# Autodesk Inventor assembly: mount_camera_static
Saved by Autodesk Inventor 2021 (Build 250183000, 183)
## iProperties
Created: 2021-03-20
Part Number: mount_camera_static
Document SubType Name: Assembly
Designer: Tomasz Lisowski
Author: Tomasz Lisowski
## Documents named in this file (5)
- T:\repos\tcodev\tco-cad\mount_camera_static\mount_camera_static.iam
- T:\repos\tcodev\tco-cad\mount_camera_static\mount_camera_static_base.ipt
- T:\repos\tcodev\tco-cad\common\coral_camera.ipt
- T:\repos\tcodev\tco-cad\common\hardware\m2_standoff_6mm.ipt
- T:\repos\tcodev\tco-cad\common\hardware\m2_bolt_cheese_5mm.ipt
## Components (14 placed, 4 different names)
1. mount_camera_static_base:1 — Rigid:1, Rigid:3, Rigid:4, Rigid:10, Rigid:11, Rigid:12, Rigid:13
2. coral_camera:1 — Rigid:14, Rigid:15, Rigid:16, Rigid:17, Rigid:18
3. m2_standoff_6mm:1 — Rigid:1
4. m2_standoff_6mm:2 — Rigid:4
5. m2_standoff_6mm:3 — Rigid:3, Rigid:14
6. m2_standoff_6mm:4
7. m2_bolt_cheese_5mm:1 — Rigid:16
8. m2_bolt_cheese_5mm:2 — Rigid:15
9. m2_bolt_cheese_5mm:3 — Rigid:17
10. m2_bolt_cheese_5mm:4 — Rigid:18
11. m2_bolt_cheese_5mm:5 — Rigid:13
12. m2_bolt_cheese_5mm:6 — Rigid:12
13. m2_bolt_cheese_5mm:7 — Rigid:11
14. m2_bolt_cheese_5mm:8 — Rigid:10
## Relationships (12: WeldJoint 12)
- Rigid:1 [WeldJoint]: mount_camera_static_base:1 ↔ m2_standoff_6mm:1
- Rigid:3 [WeldJoint]: mount_camera_static_base:1 ↔ m2_standoff_6mm:3
- Rigid:4 [WeldJoint]: mount_camera_static_base:1 ↔ m2_standoff_6mm:2
- Rigid:10 [WeldJoint]: mount_camera_static_base:1 ↔ m2_bolt_cheese_5mm:8
- Rigid:11 [WeldJoint]: mount_camera_static_base:1 ↔ m2_bolt_cheese_5mm:7
- Rigid:12 [WeldJoint]: mount_camera_static_base:1 ↔ m2_bolt_cheese_5mm:6
- Rigid:13 [WeldJoint]: mount_camera_static_base:1 ↔ m2_bolt_cheese_5mm:5
- Rigid:14 [WeldJoint]: coral_camera:1 ↔ m2_standoff_6mm:3
- Rigid:15 [WeldJoint]: coral_camera:1 ↔ m2_bolt_cheese_5mm:2
- Rigid:16 [WeldJoint]: coral_camera:1 ↔ m2_bolt_cheese_5mm:1
- Rigid:17 [WeldJoint]: coral_camera:1 ↔ m2_bolt_cheese_5mm:3
- Rigid:18 [WeldJoint]: coral_camera:1 ↔ m2_bolt_cheese_5mm:4
